# Autodesk Inventor assembly: M178-4000
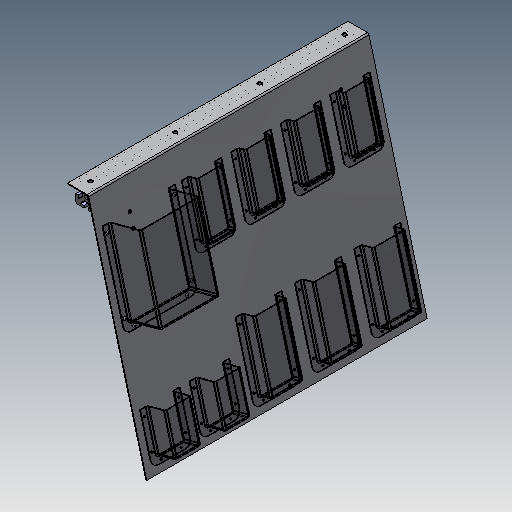
[picture p0: Inventor's stored thumbnail of the model, 512x512]
Saved by Autodesk Inventor 2018.3 (Build 223284000, 284)
## iProperties
Created: 2004-11-29
Part Number: M178-4000
Document SubType Name: Assembly
Designer: Autodesk, Inc.
Manufacturer: Standard
Standards Organization: Custom
Description: TOOL CADDY
Mass: 1512.37 g
Surface Area: 9103.48 cm^2
Volume: 746.122 cm^3
Density: 2.02698 g/cm^3
CAGE: 1LJX3
Dept. ID: Product Design
Description #2: ---
Finish #1: ---
Finish #2: ---
Material ID: ---
Project Number: ---
Author: Autodesk, Inc.
## Documents named in this file (13)
- C:\AVAInvAPI\Workspace\Test Station\Components\M178-4000.iam
- C:\AVAInvAPI\Workspace\Test Station\Components\Tool Cady Ref Mount Bar.ipt
- C:\AVAInvAPI\Workspace\Test Station\Components\M178-4002.ipt
- C:\AVAInvAPI\Workspace\Test Station\Components\MS20470 A 4-5.ipt
- C:\AVAInvAPI\Workspace\Test Station\Components\M178-4001-11.ipt
- C:\AVAInvAPI\Workspace\Test Station\Components\M178-4001-09.ipt
- C:\AVAInvAPI\Workspace\Test Station\Components\M178-4003.ipt
- C:\AVAInvAPI\Workspace\Test Station\Components\M178-4001-01.ipt
- C:\AVAInvAPI\Workspace\Test Station\Components\M178-4001-07.ipt
- C:\AVAInvAPI\Workspace\Test Station\Components\M178-4001-03.ipt
- C:\Users\kelleyb.ADS\Desktop\Samples MIGRATED 2009 224 RTM_1\Standard Parts\Test Station Content\Extrusions\40 Series Profiles.ipt
- C:\Users\kelleyb.ADS\Desktop\Samples MIGRATED 2009 224 RTM_1\Models\Assemblies\Test Station\Components\Parts\M178-4001-XX.ipt
- C:\Users\kelleyb.ADS\Desktop\Samples MIGRATED 2009 224 RTM_1\Standard Parts\Test Station Content\Rivets\MS204xx Rivets.ipt
## Components (24 placed, 9 different names)
1. Tool Cady Ref Mount Bar:1 — Flush:1, Flush:2
2. M178-4002:1 — Flush:1, Flush:2, Flush:3, Insert:1, Insert:2, Insert:8, Insert:9, Insert:12, Insert:13, Insert:14, Insert:15, Insert:16, Insert:17, Insert:24, Insert:25
3. M178-4001-07:1 — Insert:8, Insert:9
4. M178-4001-11:6 — Insert:1, Insert:2, Insert:18, Insert:19, Insert:20, Insert:21, Insert:22, Insert:23
5. MS20470 A 4-5:1 — Insert:18
6. MS20470 A 4-5:2 — Insert:19
7. MS20470 A 4-5:3 — Insert:23
8. MS20470 A 4-5:4 — Insert:22
9. MS20470 A 4-5:5 — Insert:20
10. MS20470 A 4-5:6 — Insert:21
11. M178-4003:1 — Insert:26, Insert:27
12. MS20470 A 4-5:8 — Insert:24, Insert:26
13. MS20470 A 4-5:7 — Insert:25, Insert:27
14. M178-4003:3
15. MS20470 A 4-5:9
16. MS20470 A 4-5:10
17. M178-4001-03:7 — Insert:16, Insert:17
18. M178-4001-03:2
19. M178-4001-03:3
20. M178-4001-01:8 — Insert:12, Insert:13
21. M178-4001-01:9
22. M178-4001-09:10 — Insert:14, Insert:15
23. M178-4001-09:4
24. M178-4001-09:5
## Component patterns: (2 elements, first: M178-4003:1 + MS20470 A 4-5:8 + MS20470 A 4-5:7), (4 elements, first: M178-4001-03:7), (2 elements, first: M178-4001-01:8), (3 elements, first: M178-4001-09:10)
## Relationships (23: Insert 20, Flush 3)
- Flush:1: Tool Cady Ref Mount Bar:1 ↔ M178-4002:1
- Flush:2: Tool Cady Ref Mount Bar:1 ↔ M178-4002:1
- Flush:3: M178-4002:1
- Insert:1: M178-4002:1 ↔ M178-4001-11:6
- Insert:2: M178-4002:1 ↔ M178-4001-11:6
- Insert:8: M178-4002:1 ↔ M178-4001-07:1
- Insert:9: M178-4002:1 ↔ M178-4001-07:1
- Insert:12: M178-4002:1 ↔ M178-4001-01:8
- Insert:13: M178-4002:1 ↔ M178-4001-01:8
- Insert:14: M178-4002:1 ↔ M178-4001-09:10
- Insert:15: M178-4002:1 ↔ M178-4001-09:10
- Insert:16: M178-4002:1 ↔ M178-4001-03:7
- Insert:17: M178-4002:1 ↔ M178-4001-03:7
- Insert:18: M178-4001-11:6 ↔ MS20470 A 4-5:1
- Insert:19: M178-4001-11:6 ↔ MS20470 A 4-5:2
- Insert:20: M178-4001-11:6 ↔ MS20470 A 4-5:5
- Insert:21: M178-4001-11:6 ↔ MS20470 A 4-5:6
- Insert:22: M178-4001-11:6 ↔ MS20470 A 4-5:4
- Insert:23: M178-4001-11:6 ↔ MS20470 A 4-5:3
- Insert:24: M178-4002:1 ↔ MS20470 A 4-5:8
- Insert:25: M178-4002:1 ↔ MS20470 A 4-5:7
- Insert:26: M178-4003:1 ↔ MS20470 A 4-5:8
- Insert:27: M178-4003:1 ↔ MS20470 A 4-5:7
